# Autodesk Inventor assembly: bumper_MIR
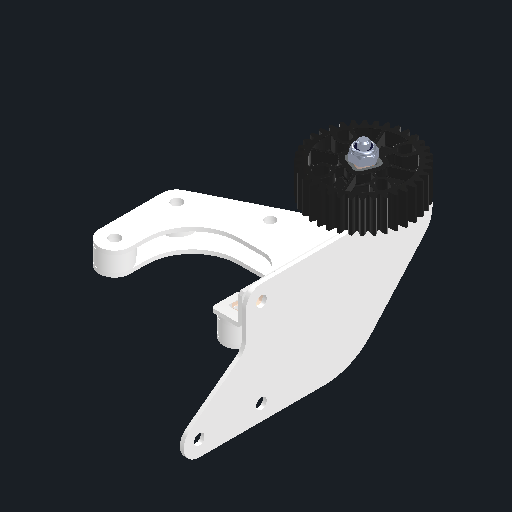
[picture p0: Inventor's stored thumbnail of the model, 512x512]
Saved by Autodesk Inventor 2024 (Build 280153000, 153)
## iProperties
Created: 2024-01-15
Part Number: bumper_MIR
Document SubType Name: Assembly
Designer: avere
Author: avere
## Documents named in this file (13)
- C:\Users\avere\Documents\rbp_cad\zoomba_v0.3\chassis\mirrored_parts\bumper_MIR.iam
- C:\Users\avere\Documents\rbp_cad\zoomba_v0.3\chassis\mirrored_parts\gusset_MIR.ipt
- C:\Users\avere\Documents\rbp_cad\VEX-CAD-Inventor-1.41\Motion\Spacers\Spacer Nylon .500 OD\NSpacer White .500 OD x .250.ipt
- C:\Users\avere\Documents\rbp_cad\VEX-CAD-Inventor-1.41\Motion\Spacers\Spacer Nylon .500 OD.ipt
- C:\Users\avere\Documents\rbp_cad\zoomba_v0.3\chassis\mirrored_parts\Alu Angle 1x1x6_MIR.ipt
- C:\Users\avere\Documents\rbp_cad\zoomba_v0.3\chassis\mirrored_parts\sled_MIR.ipt
- C:\Users\avere\Documents\rbp_cad\zoomba_v0.3\chassis\mirrored_parts\HS 36T Gear, No Insert_MIR.iam
- C:\Users\avere\Documents\rbp_cad\VEX-CAD-Inventor-1.41\Structure\Hardware\Screw Steel - Star\SScrew Star Smooth 1.750.ipt
- C:\Users\avere\Documents\rbp_cad\VEX-CAD-Inventor-1.41\Structure\Hardware\Screw Steel - Star.ipt
- C:\Users\avere\Documents\rbp_cad\zoomba_v0.3\chassis\mirrored_parts\Nut Keps_MIR.ipt
- C:\Users\avere\Documents\rbp_cad\VEX-CAD-Inventor-1.41\Motion\Spacers\Spacer Nylon .375 OD\NSpacer .375 OD x .375.ipt
- C:\Users\avere\Documents\rbp_cad\VEX-CAD-Inventor-1.41\Motion\Spacers\Spacer Nylon .375 OD.ipt
- C:\Users\avere\Documents\rbp_cad\zoomba_v0.3\chassis\mirrored_parts\Nut Thin Nylock_MIR.ipt
## Components (15 placed, 9 different names)
1. gusset_MIR:1 — Insert:2, Insert:1, Insert:5, Insert:7, Insert:9, Insert:14
2. gusset_MIR:2 — Insert:4, Insert:3, Insert:6, Insert:8, Insert:10, Mate:1, Insert:11
3. NSpacer White .500 OD x .250:1 — Insert:4, Insert:2
4. NSpacer White .500 OD x .250:2 — Insert:3, Insert:1
5. NSpacer White .500 OD x .250:3 — Insert:6, Insert:5
6. NSpacer White .500 OD x .250:4 — Insert:8, Insert:7
7. NSpacer White .500 OD x .250:5 — Insert:9
8. NSpacer White .500 OD x .250:6 — Insert:10
9. Alu Angle 1x1x6_MIR:1 — Mate:1, Insert:11, Mate:2, Insert:12, Insert:15
10. sled_MIR:1 — Mate:2, Insert:12
11. HS 36T Gear, No Insert_MIR:1 [sub-assembly] — Insert:17, Insert:18
12. SScrew Star Smooth 1.750:1 — Insert:14
13. Nut Keps_MIR:1 — Insert:15, Insert:16
14. NSpacer .375 OD x .375:1 — Insert:17, Insert:16
15. Nut Thin Nylock_MIR:1 — Insert:18
## Relationships (19: Insert 17, Mate 2)
- Insert:4: gusset_MIR:2 ↔ NSpacer White .500 OD x .250:1
- Insert:2: gusset_MIR:1 ↔ NSpacer White .500 OD x .250:1
- Insert:3: gusset_MIR:2 ↔ NSpacer White .500 OD x .250:2
- Insert:1: gusset_MIR:1 ↔ NSpacer White .500 OD x .250:2
- Insert:6: gusset_MIR:2 ↔ NSpacer White .500 OD x .250:3
- Insert:5: gusset_MIR:1 ↔ NSpacer White .500 OD x .250:3
- Insert:8: gusset_MIR:2 ↔ NSpacer White .500 OD x .250:4
- Insert:7: gusset_MIR:1 ↔ NSpacer White .500 OD x .250:4
- Insert:9: gusset_MIR:1 ↔ NSpacer White .500 OD x .250:5
- Insert:10: gusset_MIR:2 ↔ NSpacer White .500 OD x .250:6
- Mate:1: gusset_MIR:2 ↔ Alu Angle 1x1x6_MIR:1
- Insert:11: gusset_MIR:2 ↔ Alu Angle 1x1x6_MIR:1
- Mate:2: Alu Angle 1x1x6_MIR:1 ↔ sled_MIR:1
- Insert:12: Alu Angle 1x1x6_MIR:1 ↔ sled_MIR:1
- Insert:14: gusset_MIR:1 ↔ SScrew Star Smooth 1.750:1
- Insert:15: Alu Angle 1x1x6_MIR:1 ↔ Nut Keps_MIR:1
- Insert:17: HS 36T Gear, No Insert_MIR:1 ↔ NSpacer .375 OD x .375:1
- Insert:16: Nut Keps_MIR:1 ↔ NSpacer .375 OD x .375:1
- Insert:18 (0.3969 mm): HS 36T Gear, No Insert_MIR:1 ↔ Nut Thin Nylock_MIR:1
